# Autodesk Inventor assembly: RailAttachmentAssemblyLeftWithoutPi
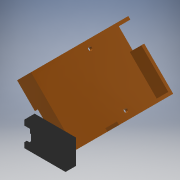
[picture p0: Inventor's stored thumbnail of the model, 180x180]
Saved by Autodesk Inventor 2018 (Build 220112000, 112)
## iProperties
Created: 2019-04-01
Part Number: RailAttachmentAssemblyLeftWithoutPi
Document SubType Name: Assembly
Designer: snipe
Author: snipe
## Documents named in this file (3)
- C:\Users\snipe\Documents\CPRE186-CAD\RailAttachmentAssemblyLeftWithoutPi.iam
- C:\Users\snipe\Documents\CPRE186-CAD\nerfRailMount.ipt
- C:\Users\snipe\Documents\CPRE186-CAD\Raspi3B+_Case.ipt
## Components (2 placed, 2 different names)
1. nerfRailMount:1 — Angle:1, Mate:7, Mate:8, Mate:9, Mate:10
2. Raspi3B+_Case:1 — Angle:1, Mate:7, Mate:8, Mate:9, Mate:10
## Relationships (5: Mate 4, Angle 1)
- Angle:1 (315 deg): nerfRailMount:1 ↔ Raspi3B+_Case:1
- Mate:7: nerfRailMount:1 ↔ Raspi3B+_Case:1
- Mate:8: nerfRailMount:1 ↔ Raspi3B+_Case:1
- Mate:9: nerfRailMount:1 ↔ Raspi3B+_Case:1
- Mate:10: nerfRailMount:1 ↔ Raspi3B+_Case:1
